# Autodesk Inventor assembly: Assembly1
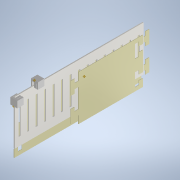
[picture p0: Inventor's stored thumbnail of the model, 180x180]
Saved by Autodesk Inventor 2021 (Build 250183000, 183)
## iProperties
Created: 2021-01-27
Part Number: Assembly1
Document SubType Name: Assembly
Designer: abij996
Author: abij996
## Documents named in this file (5)
- C:\Users\User\Documents\GitHub\2020-srw-rc-car\CoilDesign\CAD Track\Assembly1.iam
- C:\Users\phamv\OneDrive\UoA\2020 SUMMER\CAD files\primary_coil_0R2.ipt
- C:\Users\User\Documents\GitHub\2020-srw-rc-car\CoilDesign\CAD Track\Ferrite Layer\2 sections\ferrite_section.ipt
- C:\Users\User\Documents\GitHub\2020-srw-rc-car\CoilDesign\CAD Track\Top Layer\TopCoverLayer.ipt
- C:\Users\User\Documents\GitHub\2020-srw-rc-car\CoilDesign\DEXTER_WORKSPACE\CAD stuff\Final_CAD\base.ipt
## Components (11 placed, 4 different names)
1. ferrite_section:1 — Mate:1, Flush:1, Mate:2, Flush:2, Flush:3
2. ferrite_section:2 — Mate:1, Flush:1, Mate:3, Flush:4, Flush:5, Mate:7, Mate:8
3. TopCoverLayer:1 — Flush:4, Flush:5, Mate:6, Flush:9
4. TopCoverLayer:2 — Mate:4, Flush:6, Flush:7, Flush:8
5. TopCoverLayer:3 — Mate:5, Flush:8
6. TopCoverLayer:4 — Mate:6, Flush:9
7. base:1 — Mate:7
8. base:2 — Mate:8
9. TopCoverLayer:5
10. primary_coil_0R2:1 — Mate:2, Flush:2, Flush:3, Mate:3, Mate:4, Flush:6, Flush:7, Mate:5
11. primary_coil_0R2:2
## Component patterns: (2 elements, first: primary_coil_0R2:1)
## Relationships (17: Flush 9, Mate 8)
- Mate:1: ferrite_section:1 ↔ ferrite_section:2
- Flush:1: ferrite_section:1 ↔ ferrite_section:2
- Mate:2: ferrite_section:1 ↔ primary_coil_0R2:1
- Flush:2: ferrite_section:1 ↔ primary_coil_0R2:1
- Flush:3: ferrite_section:1 ↔ primary_coil_0R2:1
- Mate:3: ferrite_section:2 ↔ primary_coil_0R2:1
- Flush:4: ferrite_section:2 ↔ TopCoverLayer:1
- Flush:5: ferrite_section:2 ↔ TopCoverLayer:1
- Mate:4: TopCoverLayer:2 ↔ primary_coil_0R2:1
- Flush:6: TopCoverLayer:2 ↔ primary_coil_0R2:1
- Flush:7: TopCoverLayer:2 ↔ primary_coil_0R2:1
- Mate:5: TopCoverLayer:3 ↔ primary_coil_0R2:1
- Flush:8: TopCoverLayer:2 ↔ TopCoverLayer:3
- Mate:6: TopCoverLayer:1 ↔ TopCoverLayer:4
- Flush:9: TopCoverLayer:1 ↔ TopCoverLayer:4
- Mate:7: ferrite_section:2 ↔ base:1
- Mate:8: ferrite_section:2 ↔ base:2
